# Autodesk Inventor assembly: WholeRobotAssembly
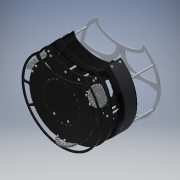
[picture p0: Inventor's stored thumbnail of the model, 180x180]
Saved by Autodesk Inventor 2017 (Build 210142000, 142)
## iProperties
Created: 2019-06-27
Part Number: WholeRobotAssembly
Document SubType Name: Assembly
Designer: cresswnd
Author: cresswnd
## Documents named in this file (18)
- C:\Users\cresswnd\Desktop\Generation 4\WholeRobotAssembly.iam
- C:\Users\cresswnd\Desktop\Generation 4\1stPlate.ipt
- C:\Users\cresswnd\Desktop\Generation 4\2ndPlate.ipt
- C:\Users\cresswnd\Desktop\Generation 4\Motor&MotorMount.iam
- C:\Users\cresswnd\Desktop\Generation 4\15mmStandoff.ipt
- C:\Users\cresswnd\Desktop\Generation 4\3rdPlate.ipt
- C:\Users\cresswnd\Desktop\Generation 4\4thPlate.ipt
- C:\Users\cresswnd\Desktop\Generation 4\Handle.ipt
- C:\Users\cresswnd\Desktop\Generation 4\19mmStandoff.ipt
- C:\Users\cresswnd\Desktop\Generation 4\8mmStandoff.ipt
- C:\Users\cresswnd\Desktop\Generation 4\3rdFront.ipt
- C:\Users\cresswnd\Desktop\Generation 4\LightGate.ipt
- C:\Users\cresswnd\Desktop\Generation 4\50mm OmniWheel Mockup.ipt
- C:\Users\cresswnd\Desktop\Generation 4\5mmScrew.ipt
- C:\Users\cresswnd\Desktop\Generation 4\2x6mmScrew.ipt
- C:\Users\cresswnd\Desktop\Generation 4\MirrorMountTest.ipt
- C:\Users\cresswnd\Desktop\Generation 4\3rdShroud.ipt
- C:\Users\cresswnd\Documents\Robotics\Version 3\Concept_1\V2\IRShroudV2.ipt
## Components (118 placed, 17 different names)
1. 1stPlate:1 — Insert:1, Insert:2, Insert:3, Insert:4, Insert:5, Insert:6, Insert:61, Insert:63, Insert:73, Insert:74, Insert:75, Insert:76, Insert:77, Insert:78, Insert:79, Insert:80
2. Motor&MotorMount:1 [sub-assembly] — Insert:1, Insert:2, Insert:7, Insert:72
3. Motor&MotorMount:2 [sub-assembly] — Insert:3, Insert:4, Insert:71
4. Motor&MotorMount:3 [sub-assembly] — Insert:5, Insert:6, Insert:8, Insert:70
5. 50mm OmniWheel Mockup:1 — Insert:72
6. 50mm OmniWheel Mockup:2 — Insert:70
7. 50mm OmniWheel Mockup:3 — Insert:71
8. 2ndPlate:1 — Insert:7, Insert:8, Insert:9, Insert:11, Insert:13, Insert:15, Insert:17, Insert:19, Insert:68, Insert:69, Insert:81, Insert:82, Insert:83, Insert:84, Insert:85, Insert:86, Insert:87, Insert:88, Insert:89, Insert:90, Insert:91, Insert:92, Insert:93, Insert:94, Insert:95, Insert:96, Insert:97, Insert:98
9. LightGate:1 — Insert:68, Insert:69
10. 3rdPlate:1 — Insert:21, Insert:22, Insert:23, Insert:25, Insert:27, Insert:29, Insert:31, Insert:33, Insert:35, Flush:2, Flush:3, Insert:99, Insert:100, Insert:102, Insert:103, Insert:111, Insert:112, Insert:121, Flush:4, Insert:132
11. IRShroudV2:1 — Insert:132
12. 3rdFront:1 — Flush:2, Flush:3, Insert:101, Insert:104, Flush:5, Insert:127, Insert:128, Insert:130, Insert:131
13. 3rdShroud:1 — Flush:4, Flush:5
14. 4thPlate:1 — Insert:37, Insert:38, Insert:39, Insert:43, Insert:47, Insert:51, Insert:105, Insert:106, Insert:107, Insert:108, Insert:109, Insert:110, Insert:113, Insert:114, Insert:115, Insert:116, Insert:122
15. MirrorMountTest:1 — Insert:123, Insert:124
16. Handle:1 — Insert:65, Insert:66, Insert:117, Insert:118, Insert:119, Insert:120, Insert:123, Insert:124, Insert:125, Insert:126
17. 5mmScrew:51 — Insert:128
18. 5mmScrew:52 — Insert:131
19. 5mmScrew:53 — Insert:130
20. 5mmScrew:54 — Insert:127
21. 5mmScrew:1 — Insert:90
22. 5mmScrew:2 — Insert:91
23. 5mmScrew:3 — Insert:94
24. 5mmScrew:4 — Insert:93
25. 5mmScrew:5 — Insert:96
26. 5mmScrew:6 — Insert:85
27. 5mmScrew:7 — Insert:98
28. 5mmScrew:8 — Insert:103
29. 5mmScrew:9 — Insert:104
30. 5mmScrew:10 — Insert:112
31. 5mmScrew:11 — Insert:109
32. 5mmScrew:12 — Insert:108
33. 5mmScrew:13 — Insert:89
34. 5mmScrew:14 — Insert:88
35. 5mmScrew:15 — Insert:115
36. 5mmScrew:16 — Insert:111
37. 5mmScrew:17 — Insert:116
38. 5mmScrew:18 — Insert:84
39. 5mmScrew:19 — Insert:83
40. 5mmScrew:20 — Insert:92
41. 5mmScrew:21 — Insert:86
42. 5mmScrew:22 — Insert:95
43. 5mmScrew:23 — Insert:87
44. 5mmScrew:24 — Insert:97
45. 5mmScrew:25 — Insert:99
46. 5mmScrew:26 — Insert:107
47. 5mmScrew:27 — Insert:102
48. 5mmScrew:28 — Insert:110
49. 5mmScrew:29 — Insert:113
50. 5mmScrew:30 — Insert:114
51. 5mmScrew:31 — Insert:106
52. 5mmScrew:32 — Insert:82
53. 5mmScrew:33 — Insert:73
54. 5mmScrew:34 — Insert:81
55. 5mmScrew:35 — Insert:74
56. 5mmScrew:36 — Insert:76
57. 5mmScrew:37 — Insert:75
58. 5mmScrew:38 — Insert:80
59. 5mmScrew:39 — Insert:77
60. 5mmScrew:40 — Insert:79
61. 5mmScrew:41 — Insert:78
62. 5mmScrew:42 — Insert:101
63. 5mmScrew:43 — Insert:100
64. 5mmScrew:44 — Insert:105
65. 5mmScrew:45 — Insert:120
66. 5mmScrew:46 — Insert:118
67. 5mmScrew:47 — Insert:119
68. 5mmScrew:48 — Insert:117
69. 2x6mmScrew:1 — Insert:125
70. 2x6mmScrew:2 — Insert:126
71. 5mmScrew:49 — Insert:121
72. 5mmScrew:50 — Insert:122
73. 15mmStandoff:1 — Insert:9, Insert:10
74. 15mmStandoff:2 — Insert:10, Insert:22
75. 15mmStandoff:3 — Insert:12, Insert:21
76. 15mmStandoff:4 — Insert:11, Insert:12
77. 15mmStandoff:5 — Insert:13, Insert:14
78. 15mmStandoff:6 — Insert:15, Insert:16
79. 15mmStandoff:7 — Insert:14
80. 15mmStandoff:8 — Insert:16
81. 15mmStandoff:9 — Insert:18
82. 15mmStandoff:10 — Insert:17, Insert:18
83. 15mmStandoff:11 — Insert:20
84. 15mmStandoff:12 — Insert:19, Insert:20
85. 15mmStandoff:13 — Insert:29, Insert:30
86. 15mmStandoff:14 — Insert:30, Insert:38
87. 15mmStandoff:15 — Insert:31, Insert:32
88. 15mmStandoff:16 — Insert:32, Insert:37
89. 15mmStandoff:17 — Insert:33, Insert:34
90. 15mmStandoff:18 — Insert:34
91. 15mmStandoff:19 — Insert:35, Insert:36
92. 15mmStandoff:20 — Insert:36
93. 15mmStandoff:21 — Insert:24
94. 15mmStandoff:22 — Insert:23, Insert:24
95. 15mmStandoff:23 — Insert:28
96. 15mmStandoff:24 — Insert:27, Insert:28
97. 15mmStandoff:25 — Insert:26
98. 15mmStandoff:26 — Insert:25, Insert:26
99. 15mmStandoff:27 — Insert:50, Insert:65
100. 15mmStandoff:28 — Insert:49, Insert:50
101. 15mmStandoff:29 — Insert:48, Insert:49
102. 15mmStandoff:30 — Insert:47, Insert:48
103. 15mmStandoff:31 — Insert:54
104. 15mmStandoff:32 — Insert:53, Insert:54
105. 15mmStandoff:33 — Insert:52, Insert:53
106. 15mmStandoff:34 — Insert:51, Insert:52
107. 15mmStandoff:35 — Insert:46
108. 15mmStandoff:36 — Insert:45, Insert:46
109. 15mmStandoff:37 — Insert:44, Insert:45
110. 15mmStandoff:38 — Insert:43, Insert:44
111. 15mmStandoff:39 — Insert:42, Insert:66
112. 15mmStandoff:40 — Insert:41, Insert:42
113. 15mmStandoff:41 — Insert:40, Insert:41
114. 15mmStandoff:42 — Insert:39, Insert:40
115. 19mmStandoff:1 — Insert:63, Insert:64
116. 19mmStandoff:3 — Insert:61, Insert:62
117. 8mmStandoff:1 — Insert:64
118. 8mmStandoff:2 — Insert:62
## Relationships (128: Insert 124, Flush 4)
- Insert:1: 1stPlate:1 ↔ Motor&MotorMount:1
- Insert:2: 1stPlate:1 ↔ Motor&MotorMount:1
- Insert:3: 1stPlate:1 ↔ Motor&MotorMount:2
- Insert:4: 1stPlate:1 ↔ Motor&MotorMount:2
- Insert:5: 1stPlate:1 ↔ Motor&MotorMount:3
- Insert:6: 1stPlate:1 ↔ Motor&MotorMount:3
- Insert:7: Motor&MotorMount:1 ↔ 2ndPlate:1
- Insert:8: Motor&MotorMount:3 ↔ 2ndPlate:1
- Insert:9: 2ndPlate:1 ↔ 15mmStandoff:1
- Insert:10: 15mmStandoff:1 ↔ 15mmStandoff:2
- Insert:11: 2ndPlate:1 ↔ 15mmStandoff:4
- Insert:12: 15mmStandoff:3 ↔ 15mmStandoff:4
- Insert:13: 2ndPlate:1 ↔ 15mmStandoff:5
- Insert:14: 15mmStandoff:5 ↔ 15mmStandoff:7
- Insert:15: 2ndPlate:1 ↔ 15mmStandoff:6
- Insert:16: 15mmStandoff:6 ↔ 15mmStandoff:8
- Insert:17: 2ndPlate:1 ↔ 15mmStandoff:10
- Insert:18: 15mmStandoff:9 ↔ 15mmStandoff:10
- Insert:19: 2ndPlate:1 ↔ 15mmStandoff:12
- Insert:20: 15mmStandoff:11 ↔ 15mmStandoff:12
- Insert:21: 3rdPlate:1 ↔ 15mmStandoff:3
- Insert:22: 3rdPlate:1 ↔ 15mmStandoff:2
- Insert:23: 3rdPlate:1 ↔ 15mmStandoff:22
- Insert:24: 15mmStandoff:21 ↔ 15mmStandoff:22
- Insert:25: 3rdPlate:1 ↔ 15mmStandoff:26
- Insert:26: 15mmStandoff:25 ↔ 15mmStandoff:26
- Insert:27: 3rdPlate:1 ↔ 15mmStandoff:24
- Insert:28: 15mmStandoff:23 ↔ 15mmStandoff:24
- Insert:29: 3rdPlate:1 ↔ 15mmStandoff:13
- Insert:30: 15mmStandoff:13 ↔ 15mmStandoff:14
- Insert:31: 3rdPlate:1 ↔ 15mmStandoff:15
- Insert:32: 15mmStandoff:15 ↔ 15mmStandoff:16
- Insert:33: 3rdPlate:1 ↔ 15mmStandoff:17
- Insert:34: 15mmStandoff:17 ↔ 15mmStandoff:18
- Insert:35: 3rdPlate:1 ↔ 15mmStandoff:19
- Insert:36: 15mmStandoff:19 ↔ 15mmStandoff:20
- Insert:37: 4thPlate:1 ↔ 15mmStandoff:16
- Insert:38: 4thPlate:1 ↔ 15mmStandoff:14
- Insert:39: 4thPlate:1 ↔ 15mmStandoff:42
- Insert:40: 15mmStandoff:41 ↔ 15mmStandoff:42
- Insert:41: 15mmStandoff:40 ↔ 15mmStandoff:41
- Insert:42: 15mmStandoff:39 ↔ 15mmStandoff:40
- Insert:43: 4thPlate:1 ↔ 15mmStandoff:38
- Insert:44: 15mmStandoff:37 ↔ 15mmStandoff:38
- Insert:45: 15mmStandoff:36 ↔ 15mmStandoff:37
- Insert:46: 15mmStandoff:35 ↔ 15mmStandoff:36
- Insert:47: 4thPlate:1 ↔ 15mmStandoff:30
- Insert:48: 15mmStandoff:29 ↔ 15mmStandoff:30
- Insert:49: 15mmStandoff:28 ↔ 15mmStandoff:29
- Insert:50: 15mmStandoff:27 ↔ 15mmStandoff:28
- Insert:51: 4thPlate:1 ↔ 15mmStandoff:34
- Insert:52: 15mmStandoff:33 ↔ 15mmStandoff:34
- Insert:53: 15mmStandoff:32 ↔ 15mmStandoff:33
- Insert:54: 15mmStandoff:31 ↔ 15mmStandoff:32
- Insert:61: 1stPlate:1 ↔ 19mmStandoff:3
- Insert:62: 19mmStandoff:3 ↔ 8mmStandoff:2
- Insert:63: 1stPlate:1 ↔ 19mmStandoff:1
- Insert:64: 19mmStandoff:1 ↔ 8mmStandoff:1
- Insert:65: Handle:1 ↔ 15mmStandoff:27
- Insert:66: Handle:1 ↔ 15mmStandoff:39
- Flush:2: 3rdPlate:1 ↔ 3rdFront:1
- Flush:3: 3rdPlate:1 ↔ 3rdFront:1
- Insert:68: 2ndPlate:1 ↔ LightGate:1
- Insert:69: 2ndPlate:1 ↔ LightGate:1
- Insert:70: Motor&MotorMount:3 ↔ 50mm OmniWheel Mockup:2
- Insert:71: Motor&MotorMount:2 ↔ 50mm OmniWheel Mockup:3
- Insert:72: Motor&MotorMount:1 ↔ 50mm OmniWheel Mockup:1
- Insert:73: 1stPlate:1 ↔ 5mmScrew:33
- Insert:74: 1stPlate:1 ↔ 5mmScrew:35
- Insert:75: 1stPlate:1 ↔ 5mmScrew:37
- Insert:76: 1stPlate:1 ↔ 5mmScrew:36
- Insert:77: 1stPlate:1 ↔ 5mmScrew:39
- Insert:78: 1stPlate:1 ↔ 5mmScrew:41
- Insert:79: 1stPlate:1 ↔ 5mmScrew:40
- Insert:80: 1stPlate:1 ↔ 5mmScrew:38
- Insert:81: 2ndPlate:1 ↔ 5mmScrew:34
- Insert:82: 2ndPlate:1 ↔ 5mmScrew:32
- Insert:83: 2ndPlate:1 ↔ 5mmScrew:19
- Insert:84: 2ndPlate:1 ↔ 5mmScrew:18
- Insert:85: 2ndPlate:1 ↔ 5mmScrew:6
- Insert:86: 2ndPlate:1 ↔ 5mmScrew:21
- Insert:87: 2ndPlate:1 ↔ 5mmScrew:23
- Insert:88: 2ndPlate:1 ↔ 5mmScrew:14
- Insert:89: 2ndPlate:1 ↔ 5mmScrew:13
- Insert:90: 2ndPlate:1 ↔ 5mmScrew:1
- Insert:91: 2ndPlate:1 ↔ 5mmScrew:2
- Insert:92: 2ndPlate:1 ↔ 5mmScrew:20
- Insert:93: 2ndPlate:1 ↔ 5mmScrew:4
- Insert:94: 2ndPlate:1 ↔ 5mmScrew:3
- Insert:95: 2ndPlate:1 ↔ 5mmScrew:22
- Insert:96: 2ndPlate:1 ↔ 5mmScrew:5
- Insert:97: 2ndPlate:1 ↔ 5mmScrew:24
- Insert:98: 2ndPlate:1 ↔ 5mmScrew:7
- Insert:99: 3rdPlate:1 ↔ 5mmScrew:25
- Insert:100: 3rdPlate:1 ↔ 5mmScrew:43
- Insert:101: 3rdFront:1 ↔ 5mmScrew:42
- Insert:102: 3rdPlate:1 ↔ 5mmScrew:27
- Insert:103: 3rdPlate:1 ↔ 5mmScrew:8
- Insert:104: 3rdFront:1 ↔ 5mmScrew:9
- Insert:105: 4thPlate:1 ↔ 5mmScrew:44
- Insert:106: 4thPlate:1 ↔ 5mmScrew:31
- Insert:107: 4thPlate:1 ↔ 5mmScrew:26
- Insert:108: 4thPlate:1 ↔ 5mmScrew:12
- Insert:109: 4thPlate:1 ↔ 5mmScrew:11
- Insert:110: 4thPlate:1 ↔ 5mmScrew:28
- Insert:111: 3rdPlate:1 ↔ 5mmScrew:16
- Insert:112: 3rdPlate:1 ↔ 5mmScrew:10
- Insert:113: 4thPlate:1 ↔ 5mmScrew:29
- Insert:114: 4thPlate:1 ↔ 5mmScrew:30
- Insert:115: 4thPlate:1 ↔ 5mmScrew:15
- Insert:116: 4thPlate:1 ↔ 5mmScrew:17
- Insert:117: Handle:1 ↔ 5mmScrew:48
- Insert:118: Handle:1 ↔ 5mmScrew:46
- Insert:119: Handle:1 ↔ 5mmScrew:47
- Insert:120: Handle:1 ↔ 5mmScrew:45
- Insert:121: 3rdPlate:1 ↔ 5mmScrew:49
- Insert:122: 4thPlate:1 ↔ 5mmScrew:50
- Insert:123: MirrorMountTest:1 ↔ Handle:1
- Insert:124: MirrorMountTest:1 ↔ Handle:1
- Insert:125: Handle:1 ↔ 2x6mmScrew:1
- Insert:126: Handle:1 ↔ 2x6mmScrew:2
- Flush:4: 3rdPlate:1 ↔ 3rdShroud:1
- Flush:5: 3rdFront:1 ↔ 3rdShroud:1
- Insert:127: 3rdFront:1 ↔ 5mmScrew:54
- Insert:128: 3rdFront:1 ↔ 5mmScrew:51
- Insert:130: 3rdFront:1 ↔ 5mmScrew:53
- Insert:131: 3rdFront:1 ↔ 5mmScrew:52
- Insert:132: 3rdPlate:1 ↔ IRShroudV2:1
